# Autodesk Inventor assembly: rod_assembly
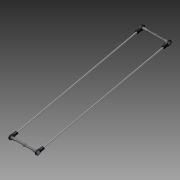
[picture p0: Inventor's stored thumbnail of the model, 180x180]
Saved by Autodesk Inventor 2012 (Build 160160000, 160)
## iProperties
Created: 2013-10-02
Part Number: rod_assembly
Document SubType Name: Assembly
Designer: Nick
Author: Nick
## Documents named in this file (4)
- C:\Users\Nick\Documents\GitHub\DeltaRobot\cad_v1\rod_assembly.iam
- C:\Users\Nick\Documents\GitHub\DeltaRobot\cad_v1\union.ipt
- C:\Users\Nick\Documents\GitHub\DeltaRobot\cad_v1\rod.ipt
- C:\Users\Nick\Documents\GitHub\DeltaRobot\cad_v1\union2.ipt
## Components (8 placed, 3 different names)
1. union:1 — Mate:9, Mate:10, Flush:2, Mate:14
2. union:2 — Mate:12, Flush:1, Mate:13, Flush:3
3. rod:1 — Insert:5, Insert:6
4. rod:2 — Insert:7, Insert:8
5. union2:1 — Mate:12, Flush:1, Insert:6
6. union2:2 — Insert:8, Mate:14
7. union2:3 — Mate:9, Mate:10, Insert:5, Flush:2
8. union2:4 — Mate:13, Insert:7, Flush:3
## Relationships (12: Mate 5, Insert 4, Flush 3)
- Mate:9: union:1 ↔ union2:3
- Mate:10: union:1 ↔ union2:3
- Insert:5 (-3 mm): rod:1 ↔ union2:3
- Mate:12: union:2 ↔ union2:1
- Flush:1 (0.5 mm): union:2 ↔ union2:1
- Flush:2 (0.5 mm): union:1 ↔ union2:3
- Insert:6 (-3 mm): rod:1 ↔ union2:1
- Mate:13: union:2 ↔ union2:4
- Insert:7 (-3 mm): rod:2 ↔ union2:4
- Flush:3 (0.5 mm): union:2 ↔ union2:4
- Insert:8 (-3 mm): rod:2 ↔ union2:2
- Mate:14: union:1 ↔ union2:2
